# Autodesk Inventor assembly: Assembly_0_scooter_visual
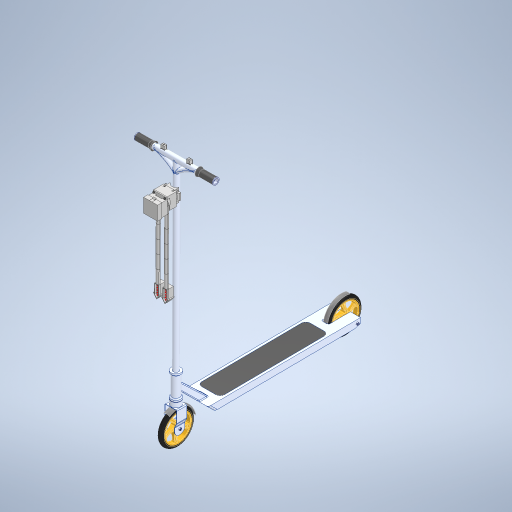
[picture p0: Inventor's stored thumbnail of the model, 512x512]
Saved by Autodesk Inventor 2023 (Build 270158000, 158)
## iProperties
Created: 2023-10-25
Part Number: Assembly_0_scooter_visual
Document SubType Name: Assembly
Designer: zskus
Author: zskus
## Documents named in this file (4)
- C:\Users\zskus\Desktop\Folders\Personal Projects\Inventor\Project_1_Scooter\Assembly\Assembly_0_scooter_visual.iam
- C:\Users\zskus\Desktop\Folders\Personal Projects\Inventor\Project_1_Scooter\Kick Scooter\Assembly.iam
- C:\Users\zskus\Desktop\Folders\Personal Projects\Inventor\Project_1_Scooter\Assembly\Assembly_3_master.iam
- C:\Users\zskus\Desktop\Folders\Personal Projects\Inventor\Project_1_Scooter\Assembly\Assembly_7_button.iam
## Components (4 placed, 3 different names)
1. Assembly:1 [sub-assembly] — Mate:1, Mate:2, Mate:3, Mate:4, Mate:5
2. Assembly_3_master:1 [sub-assembly] — Mate:1, Angle:1, Flush:1
3. Assembly_7_button:1 [sub-assembly] — Mate:2, Angle:3, Mate:5
4. Assembly_7_button:2 [sub-assembly] — Mate:3, Angle:2, Mate:4
## Relationships (9: Mate 5, Angle 3, Flush 1)
- Mate:1: Assembly:1 ↔ Assembly_3_master:1
- Angle:1 (180 deg): Assembly_3_master:1
- Flush:1 (-127 mm): Assembly_3_master:1
- Mate:2: Assembly:1 ↔ Assembly_7_button:1
- Mate:3: Assembly:1 ↔ Assembly_7_button:2
- Angle:2 (180 deg): Assembly_7_button:2
- Angle:3 (180 deg): Assembly_7_button:1
- Mate:4 (50.8 mm): Assembly:1 ↔ Assembly_7_button:2
- Mate:5 (50.8 mm): Assembly:1 ↔ Assembly_7_button:1
